# Autodesk Inventor assembly: Ass_fiqh
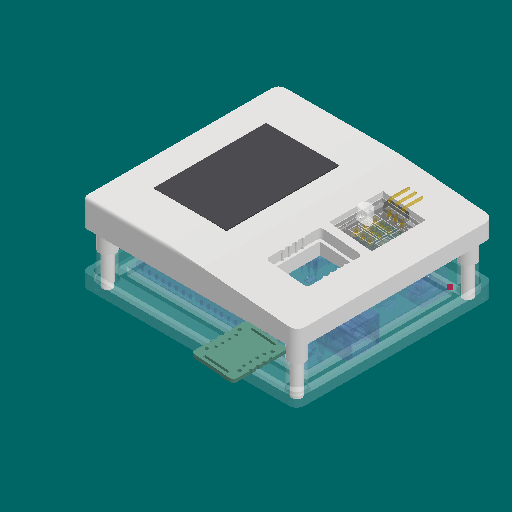
[picture p0: Inventor's stored thumbnail of the model, 512x512]
Saved by Autodesk Inventor 2025.2 (Build 292293000, 293)
## iProperties
Created: 2025-05-06
Part Number: Ass_fiqh
Document SubType Name: Assembly
Designer: ia088
Author: ia088
## Documents named in this file (7)
- C:\Users\ia088\OneDrive\Dokumen\fiqhin\Ass_fiqh.iam
- C:\Users\ia088\OneDrive\Dokumen\fiq\arduino-uno-r3-1.snapshot.5\arduino uno\arduino uno\arduino uno.ipt
- C:\Users\ia088\OneDrive\Dokumen\fiq\MAX30102_MH_ET_LIVE_BOARD_v8\MAX30102_MH_ET_LIVE_BOARD_v8\MAX30102_MH_ET_LIVE_BOARD_v8.ipt
- C:\Users\ia088\OneDrive\Dokumen\fiqhin\Part_uno_bawah.ipt
- C:\Users\ia088\OneDrive\Dokumen\fiq\1.54  i2c oled\1.54  i2c oled\1.54  i2c oled.ipt
- C:\Users\ia088\OneDrive\Dokumen\fiq\DS18B20 Module\KY-001 DS18B20 Module\KY-001 DS18B20 Module\KY-001 DS18B20 Module.ipt
- C:\Users\ia088\OneDrive\Dokumen\fiqhin\Part_uno_atas_.ipt
## Components (6 placed, 6 different names)
1. arduino uno:1 — Mate:1, Flush:1
2. Part_uno_bawah:1 — Mate:1, Flush:1, Mate:2, Mate:3, Mate:4
3. 1.54  i2c oled:1 — Mate:2, Flush:5, Mate:5
4. Part_uno_atas_:1 — Mate:3, Mate:4, Flush:5, Mate:5, Mate:6, Flush:6, Flush:7, Flush:8
5. KY-001 DS18B20 Module:1 — Mate:6, Flush:6, Flush:7
6. MAX30102_MH_ET_LIVE_BOARD_v8:1 — Flush:8
## Relationships (11: Mate 6, Flush 5)
- Mate:1: arduino uno:1 ↔ Part_uno_bawah:1
- Flush:1: arduino uno:1 ↔ Part_uno_bawah:1
- Mate:2: Part_uno_bawah:1 ↔ 1.54  i2c oled:1
- Mate:3: Part_uno_bawah:1 ↔ Part_uno_atas_:1
- Mate:4: Part_uno_bawah:1 ↔ Part_uno_atas_:1
- Flush:5: 1.54  i2c oled:1 ↔ Part_uno_atas_:1
- Mate:5: 1.54  i2c oled:1 ↔ Part_uno_atas_:1
- Mate:6: Part_uno_atas_:1 ↔ KY-001 DS18B20 Module:1
- Flush:6: Part_uno_atas_:1 ↔ KY-001 DS18B20 Module:1
- Flush:7: Part_uno_atas_:1 ↔ KY-001 DS18B20 Module:1
- Flush:8: Part_uno_atas_:1 ↔ MAX30102_MH_ET_LIVE_BOARD_v8:1
